# Autodesk Inventor assembly: DividerAssembly
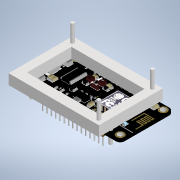
[picture p0: Inventor's stored thumbnail of the model, 180x180]
Saved by Autodesk Inventor 2021 (Build 250183000, 183)
## iProperties
Created: 2023-10-10
Part Number: DividerAssembly
Document SubType Name: Assembly
Designer: 21seblin
Author: 21seblin
## Documents named in this file (3)
- C:\Users\21seblin\Documents\GitHub\MDU-SamarbetanderobotarDVA138\Projekt\Inventor-CAD\DividerAssembly.iam
- C:\Users\21seblin\Documents\GitHub\MDU-SamarbetanderobotarDVA138\Projekt\Inventor-CAD\Divider_NodeMCU_Sipeed.ipt
- C:\Users\21seblin\Downloads\ESP8266.ipt
## Components (2 placed, 2 different names)
1. Divider_NodeMCU_Sipeed:1 — Mate:1, Mate:2
2. ESP8266:1 — Mate:1, Mate:2
## Relationships (2: Mate 2)
- Mate:1: Divider_NodeMCU_Sipeed:1 ↔ ESP8266:1
- Mate:2: Divider_NodeMCU_Sipeed:1 ↔ ESP8266:1
